# Autodesk Inventor assembly: Pick_&_Place_Nozzle_Assembly
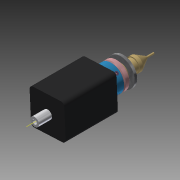
[picture p0: Inventor's stored thumbnail of the model, 180x180]
Saved by Autodesk Inventor 2015 (Build 190159000, 159)
## iProperties
Created: 2015-01-06
Part Number: Pick_&_Place_Nozzle_Assembly
Document SubType Name: Assembly
Designer: ice
Author: ice
## Documents named in this file (4)
- C:\Users\ice\Documents\GitHub\PnP-Magnetic-Tool-Tip\Inventor\Pick_&_Place_Nozzle_Assembly_Nozzle_#2.iam
- C:\Users\ice\Documents\GitHub\PnP-Magnetic-Tool-Tip\Inventor\NEMA8.ipt
- C:\Users\ice\Documents\GitHub\PnP-Magnetic-Tool-Tip\Inventor\Magnetic_Extender_Assembly.iam
- C:\Users\ice\Documents\GitHub\PnP-Magnetic-Tool-Tip\Inventor\Assembly_Nozzle_#2.iam
## Components (3 placed, 3 different names)
1. NEMA8:1 — Mate:16, Mate:17
2. Magnetic_Extender_Assembly:1 [sub-assembly] — Mate:16, Mate:17, Mate:18, Mate:19
3. Assembly_Nozzle_#2:1 [sub-assembly] — Mate:18, Mate:19
## Relationships (4: Mate 4)
- Mate:16: NEMA8:1 ↔ Magnetic_Extender_Assembly:1
- Mate:17: NEMA8:1 ↔ Magnetic_Extender_Assembly:1
- Mate:18: Magnetic_Extender_Assembly:1 ↔ Assembly_Nozzle_#2:1
- Mate:19: Magnetic_Extender_Assembly:1 ↔ Assembly_Nozzle_#2:1
